# Autodesk Inventor assembly: mikrosumo
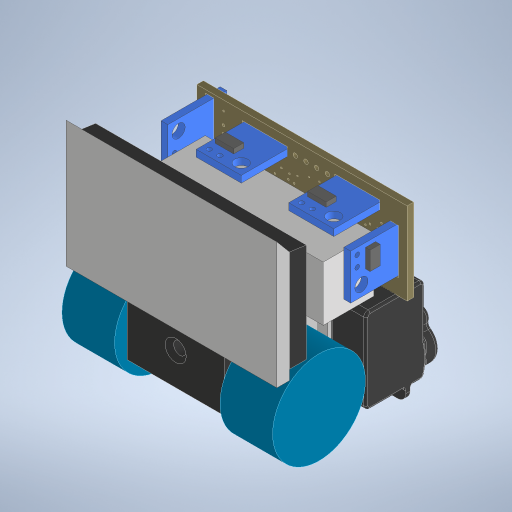
[picture p0: Inventor's stored thumbnail of the model, 512x512]
Saved by Autodesk Inventor 2023 (Build 270158000, 158)
## iProperties
Created: 2022-12-13
Part Number: mikrosumo
Document SubType Name: Assembly
Designer: komputer
Author: komputer
## Documents named in this file (10)
- D:\Inventor\MikroSumo\mikrosumo.iam
- D:\Inventor\MikroSumo\podsta.ipt
- D:\Inventor\MikroSumo\koło.ipt
- D:\Inventor\MikroSumo\opona.ipt
- D:\Inventor\MikroSumo\pokrywa silników.ipt
- D:\Inventor\MikroSumo\lipol 150mAH.ipt
- D:\Inventor\MikroSumo\nozz.ipt
- C:\Users\Kamil\Desktop\pulpit\powerhd_hd_1370a_micro.ipt
- C:\Users\Kamil\Desktop\TOF_VLCOS.ipt
- C:\Users\Kamil\Desktop\PCB_BEETLE.iam
## Components (15 placed, 9 different names)
1. podsta:1 — Flush:1, Mate:1, Flush:2
2. koło:1
3. koło:2
4. opona:1
5. opona:2
6. lipol 150mAH:1
7. nozz:1
8. pokrywa silników:2 — Flush:1, Mate:1, Flush:2, Mate:3, Zestawiające:17, Zestawiające:18, Zestawiające:19
9. powerhd_hd_1370a_micro:1 — Mate:3, Flush:7
10. powerhd_hd_1370a_micro:2 — Flush:7
11. TOF_VLCOS:1 — Zestawiające:25, Zestawiające:26, Równoległe:13
12. TOF_VLCOS:2 — Równoległe:11, Zestawiające:20, Zestawiające:28
13. TOF_VLCOS:3 — Zestawiające:24, Zestawiające:27, Równoległe:14
14. TOF_VLCOS:5 — Równoległe:12, Zestawiające:22, Zestawiające:23
15. PCB_BEETLE:1 [sub-assembly] — Zestawiające:17, Zestawiające:18, Zestawiające:19, Równoległe:11, Zestawiające:20, Równoległe:12, Zestawiające:22, Zestawiające:23, Zestawiające:24, Zestawiające:25, Zestawiające:26, Zestawiające:27, Równoległe:13, Równoległe:14, Zestawiające:28
## Relationships (20: Mate 13, Flush 7)
- Flush:1: podsta:1 ↔ pokrywa silników:2
- Mate:1 (11.5 mm): podsta:1 ↔ pokrywa silników:2
- Flush:2: podsta:1 ↔ pokrywa silników:2
- Mate:3: pokrywa silników:2 ↔ powerhd_hd_1370a_micro:1
- Flush:7: powerhd_hd_1370a_micro:1 ↔ powerhd_hd_1370a_micro:2
- Zestawiające:17 [Mate]: pokrywa silników:2 ↔ PCB_BEETLE:1
- Zestawiające:18 [Mate]: pokrywa silników:2 ↔ PCB_BEETLE:1
- Zestawiające:19 [Mate]: pokrywa silników:2 ↔ PCB_BEETLE:1
- Równoległe:11 [Flush] (-1.5 mm): TOF_VLCOS:2 ↔ PCB_BEETLE:1
- Zestawiające:20 [Mate]: TOF_VLCOS:2 ↔ PCB_BEETLE:1
- Równoległe:12 [Flush] (-1.5 mm): TOF_VLCOS:5 ↔ PCB_BEETLE:1
- Zestawiające:22 [Mate]: TOF_VLCOS:5 ↔ PCB_BEETLE:1
- Zestawiające:23 [Mate]: TOF_VLCOS:5 ↔ PCB_BEETLE:1
- Zestawiające:24 [Mate]: TOF_VLCOS:3 ↔ PCB_BEETLE:1
- Zestawiające:25 [Mate]: TOF_VLCOS:1 ↔ PCB_BEETLE:1
- Zestawiające:26 [Mate]: TOF_VLCOS:1 ↔ PCB_BEETLE:1
- Zestawiające:27 [Mate]: TOF_VLCOS:3 ↔ PCB_BEETLE:1
- Równoległe:13 [Flush] (-1.5 mm): TOF_VLCOS:1 ↔ PCB_BEETLE:1
- Równoległe:14 [Flush] (-1.5 mm): TOF_VLCOS:3 ↔ PCB_BEETLE:1
- Zestawiające:28 [Mate]: TOF_VLCOS:2 ↔ PCB_BEETLE:1
